# Autodesk Inventor assembly: Assembly2
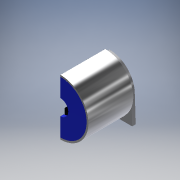
[picture p0: Inventor's stored thumbnail of the model, 180x180]
Saved by Autodesk Inventor 2017 (Build 210142000, 142)
## iProperties
Created: 2017-11-23
Part Number: Assembly2
Document SubType Name: Assembly
Designer: prakh
Author: prakh
## Documents named in this file (13)
- C:\Users\prakh\OneDrive\Documents\McMaster Year 6\capstone\Clutch Whel compat\Assembly2.iam
- C:\Users\prakh\OneDrive\Documents\McMaster Year 6\capstone\Clutch Whel compat\wheel hub.ipt
- C:\Users\prakh\OneDrive\Documents\McMaster Year 6\capstone\Clutch Whel compat\wheel ring.ipt
- C:\Users\prakh\OneDrive\Documents\McMaster Year 6\capstone\Clutch Whel compat\clutch plate.ipt
- C:\Users\prakh\OneDrive\Documents\McMaster Year 6\capstone\Clutch Whel compat\ball bearing ball 0.25in.ipt
- C:\Users\prakh\OneDrive\Documents\McMaster Year 6\capstone\Clutch Whel compat\clutch washer.ipt
- C:\Users\prakh\OneDrive\Documents\McMaster Year 6\capstone\Clutch Whel compat\mounting plate.ipt
- C:\Users\prakh\OneDrive\Documents\McMaster Year 6\capstone\Clutch Whel compat\motor mount 2.ipt
- C:\Users\prakh\OneDrive\Documents\McMaster Year 6\capstone\Clutch Whel compat\POT.ipt
- C:\Users\prakh\OneDrive\Documents\McMaster Year 6\capstone\Clutch Whel compat\Assembly2\Design Accelerator\Spur Gears1.iam
- C:\Users\prakh\OneDrive\Documents\McMaster Year 6\capstone\Clutch Whel compat\spring cap.ipt
- C:\Users\prakh\OneDrive\Documents\McMaster Year 6\capstone\Clutch Whel compat\3590s-2.ipt
- C:\Users\prakh\OneDrive\Documents\McMaster Year 6\capstone\Clutch Whel compat\Spur Gear21 pot.ipt
## Components (16 placed, 12 different names)
1. mounting plate:1 — Flush:2, Flush:3, Flush:4, Mate:16, Mate:17, Mate:18, Mate:19, Mate:20, Mate:21, Mate:22, Mate:24, Mate:25, Mate:26, Angle:1, Mate:27, Mate:28
2. wheel hub:1 — Mate:1, Flush:1, Mate:8, Mate:9, Mate:10, Mate:11, Mate:12, Mate:13
3. wheel ring:1 — Mate:1, Flush:1, Mate:2, Mate:16
4. clutch plate:1 — Mate:2, Mate:3, Mate:4, Mate:5, Mate:6, Mate:7, Mate:13, Mate:14, Mate:26
5. ball bearing ball 0.25in:1 — Mate:3, Mate:9
6. ball bearing ball 0.25in:2 — Mate:4, Mate:8, Mate:15
7. ball bearing ball 0.25in:3 — Mate:5, Mate:10
8. ball bearing ball 0.25in:4 — Mate:6, Mate:12
9. ball bearing ball 0.25in:5 — Mate:7, Mate:11
10. clutch washer:1 — Mate:14, Mate:15
11. motor mount 2:1 — Mate:17, Mate:18
12. POT:1 — Mate:19, Mate:20, Mate:23
13. Spur Gears:1 [sub-assembly] — Mate:21, Mate:22, Mate:23, Mate:24, Tangent:1, Rotation:1
14. spring cap:1 — Mate:25, Angle:1, Tangent:1
15. 3590s-2:1 — Mate:27, Mate:28, Mate:29, Mate:30
16. Spur Gear2:1 — Mate:29, Mate:30, Rotation:1
## Relationships (37: Mate 30, Flush 4, Angle 1, Tangent 1, RelateRotation 1)
- Mate:1: wheel hub:1 ↔ wheel ring:1
- Flush:1: wheel hub:1 ↔ wheel ring:1
- Mate:2: wheel ring:1 ↔ clutch plate:1
- Mate:3: clutch plate:1 ↔ ball bearing ball 0.25in:1
- Mate:4: clutch plate:1 ↔ ball bearing ball 0.25in:2
- Mate:5: clutch plate:1 ↔ ball bearing ball 0.25in:3
- Mate:6: clutch plate:1 ↔ ball bearing ball 0.25in:4
- Mate:7: clutch plate:1 ↔ ball bearing ball 0.25in:5
- Mate:8 (1.5875 mm): wheel hub:1 ↔ ball bearing ball 0.25in:2
- Mate:9 (1.5875 mm): wheel hub:1 ↔ ball bearing ball 0.25in:1
- Mate:10 (1.5875 mm): wheel hub:1 ↔ ball bearing ball 0.25in:3
- Mate:11 (1.5875 mm): wheel hub:1 ↔ ball bearing ball 0.25in:5
- Mate:12 (1.5875 mm): wheel hub:1 ↔ ball bearing ball 0.25in:4
- Mate:13 (1.5875 mm): wheel hub:1 ↔ clutch plate:1
- Mate:14: clutch plate:1 ↔ clutch washer:1
- Mate:15 (3.175 mm): ball bearing ball 0.25in:2 ↔ clutch washer:1
- Flush:2: mounting plate:1
- Flush:3: mounting plate:1
- Flush:4: mounting plate:1
- Mate:16: mounting plate:1 ↔ wheel ring:1
- Mate:17: mounting plate:1 ↔ motor mount 2:1
- Mate:18: mounting plate:1 ↔ motor mount 2:1
- Mate:19: mounting plate:1 ↔ POT:1
- Mate:20: mounting plate:1 ↔ POT:1
- Mate:21: mounting plate:1 ↔ Spur Gears:1
- Mate:22: mounting plate:1 ↔ Spur Gears:1
- Mate:23: POT:1 ↔ Spur Gears:1
- Mate:24: mounting plate:1 ↔ Spur Gears:1
- Mate:25: mounting plate:1 ↔ spring cap:1
- Mate:26 (3.175 mm): mounting plate:1 ↔ clutch plate:1
- Angle:1 (0 deg): mounting plate:1 ↔ spring cap:1
- Tangent:1: Spur Gears:1 ↔ spring cap:1
- Mate:27: mounting plate:1 ↔ 3590s-2:1
- Mate:28: mounting plate:1 ↔ 3590s-2:1
- Mate:29: 3590s-2:1 ↔ Spur Gear2:1
- Mate:30: 3590s-2:1 ↔ Spur Gear2:1
- Rotation:1 [RelateRotation] (0.199 ul): Spur Gears:1 ↔ Spur Gear2:1
